# Autodesk Inventor assembly: Modelo_Completo_3
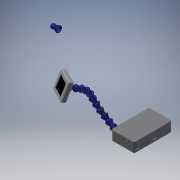
[picture p0: Inventor's stored thumbnail of the model, 180x180]
Saved by Autodesk Inventor 2019 (Build 230136000, 136)
## iProperties
Created: 2018-11-28
Part Number: Modelo_Completo_3
Material: Generic
Document SubType Name: Assembly
Designer: cadcae
Author: cadcae
## Documents named in this file (4)
- C:\Users\CADCAE\Downloads\CAD_thesis\Modelo_Completo_3.iam
- C:\Users\CADCAE\Downloads\CAD_thesis\Case_Principal_3.iam
- C:\Users\CADCAE\Downloads\CAD_thesis\Loc-line\1-4 Element.ipt
- C:\Users\CADCAE\Downloads\CAD_thesis\Case_Pantalla.iam
## Components (14 placed, 3 different names)
1. Case_Principal_3:1 [sub-assembly] — Flush:1, Flush:2, Flush:3, Ball:1
2. 1-4 Element:1 — Ball:1, Ball:2
3. 1-4 Element:2 — Ball:2, Ball:3
4. 1-4 Element:3 — Ball:3, Ball:4
5. 1-4 Element:4 — Ball:4, Ball:5
6. 1-4 Element:5 — Ball:5, Ball:6
7. 1-4 Element:6 — Ball:6, Ball:7
8. 1-4 Element:7 — Ball:7, Ball:8
9. 1-4 Element:8 — Ball:8, Ball:9
10. 1-4 Element:9 — Ball:9, Ball:10
11. 1-4 Element:10 — Ball:10, Ball:11
12. 1-4 Element:11 — Ball:11, Ball:12
13. 1-4 Element:12
14. Case_Pantalla:1 [sub-assembly] — Ball:12
## Relationships (15: BallJoint 12, Flush 3)
- Flush:1: Case_Principal_3:1
- Flush:2: Case_Principal_3:1
- Flush:3: Case_Principal_3:1
- Ball:1: Case_Principal_3:1 ↔ 1-4 Element:1
- Ball:2: 1-4 Element:1 ↔ 1-4 Element:2
- Ball:3: 1-4 Element:2 ↔ 1-4 Element:3
- Ball:4: 1-4 Element:3 ↔ 1-4 Element:4
- Ball:5: 1-4 Element:4 ↔ 1-4 Element:5
- Ball:6: 1-4 Element:5 ↔ 1-4 Element:6
- Ball:7: 1-4 Element:6 ↔ 1-4 Element:7
- Ball:8: 1-4 Element:7 ↔ 1-4 Element:8
- Ball:9: 1-4 Element:8 ↔ 1-4 Element:9
- Ball:10: 1-4 Element:9 ↔ 1-4 Element:10
- Ball:11: 1-4 Element:10 ↔ 1-4 Element:11
- Ball:12: 1-4 Element:11 ↔ Case_Pantalla:1
